# Autodesk Inventor assembly: Carrinho + Pista
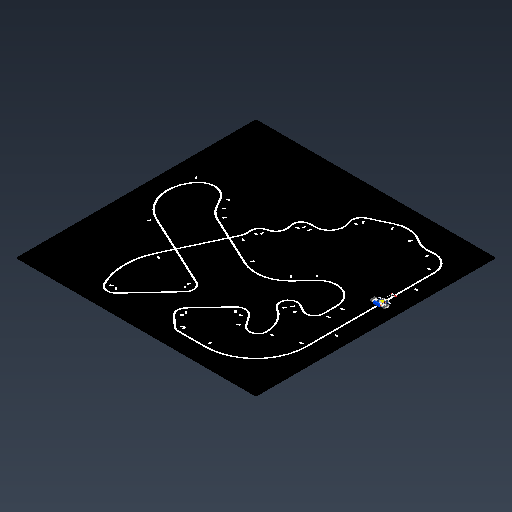
[picture p0: Inventor's stored thumbnail of the model, 512x512]
Saved by Autodesk Inventor 2026.1 (Build 301233020, 233B)
## iProperties
Created: 2026-04-04
Part Number: Carrinho + Pista
Document SubType Name: Assembly
Designer: celio
Author: celio
## Documents named in this file (3)
- C:\Users\celio\OneDrive\Documentos\Inventor\ZeGuia\Carrinho + Pista.iam
- C:\Users\celio\OneDrive\Documentos\Inventor\ZeGuia\Pista_V2.ipt
- C:\Users\celio\OneDrive\Documentos\Inventor\ZeGuia\Montagem Ze Guia.iam
## Components (2 placed, 2 different names)
1. Pista_V2:1 — Alinhado:1
2. Montagem Ze Guia:1 [sub-assembly] — Alinhado:1
## Relationships (1: Flush 1)
- Alinhado:1 [Flush]: Pista_V2:1 ↔ Montagem Ze Guia:1
